# Autodesk Inventor assembly: nano shield
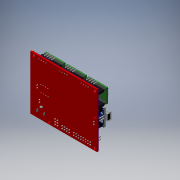
[picture p0: Inventor's stored thumbnail of the model, 180x180]
Saved by Autodesk Inventor 2018 (Build 220112000, 112)
## iProperties
Created: 2018-03-19
Part Number: nano shield
Material: Genérico
Document SubType Name: Assembly
Designer: usuario
Author: usuario
## Documents named in this file (11)
- D:\vape\modelos vape\nano arduino shield cnc\nano shield.iam
- D:\vape\modelos vape\cnc\nano.ipt
- D:\vape\modelos vape\cnc\Headers Machos\Files Inventor\PZ_header_single_1pin.ipt
- D:\vape\modelos vape\cnc\Headers Machos\Files Inventor\PZ_header14pines.ipt
- D:\vape\modelos vape\cnc\Headers Machos\Files Inventor\PZ_header_single_3pines.ipt
- D:\vape\modelos vape\cnc\Headers Machos\Files Inventor\User Library-Header 4 Vertical.ipt
- D:\vape\modelos vape\cnc\arduino-diecimila-t8730\Arduino Diecimila T8730\2.1mm DC Power Socket\2.1mm DC Power Socket.iam
- D:\vape\modelos vape\cnc\arduino-diecimila-t8730\Arduino Diecimila T8730\2.5mm Pitch Miniature Socket - Digital.ipt
- D:\vape\modelos vape\cnc\pololu.ipt
- D:\vape\modelos vape\cnc\SIL_Socket08_.iam
- D:\vape\modelos vape\cnc\arduino-nano-4.snapshot.1\Arduino Nano\Arduino Nano.ipt
## Components (34 placed, 10 different names)
1. nano:1 — Coincidencia:1, Coincidencia:2, Coincidencia:4, Coincidencia:7, Coincidencia:8, Coincidencia:10, Coincidencia:12, Coincidencia:15, Coincidencia:16, Coincidencia:18, Coincidencia:19, Nivelación:7, Coincidencia:20, Coincidencia:21, Coincidencia:25, Coincidencia:26, Coincidencia:27, Coincidencia:28, Coincidencia:29, Coincidencia:30, Coincidencia:31, Coincidencia:32, Coincidencia:33, Coincidencia:37, Coincidencia:39
2. PZ_header_single_1pin:1 — Coincidencia:1, Coincidencia:3, Nivelación:1, Coincidencia:5
3. PZ_header14pines:1 — Coincidencia:2, Coincidencia:3, Nivelación:1, Coincidencia:6, Nivelación:2
4. PZ_header_single_1pin:2 — Coincidencia:4, Coincidencia:5, Coincidencia:6
5. PZ_header_single_1pin:3 — Coincidencia:7, Nivelación:2, Coincidencia:9, Nivelación:3, Coincidencia:14
6. PZ_header_single_1pin:4 — Coincidencia:12, Coincidencia:13, Coincidencia:14
7. PZ_header_single_3pines:1 — Coincidencia:8, Coincidencia:9, Nivelación:3, Coincidencia:11, Nivelación:4, Nivelación:5
8. PZ_header_single_3pines:2 — Coincidencia:10, Coincidencia:11, Nivelación:4, Coincidencia:13
9. PZ_header_single_3pines:3 — Coincidencia:15, Nivelación:5, Nivelación:6, Coincidencia:17
10. PZ_header_single_3pines:4 — Coincidencia:16, Nivelación:6, Coincidencia:17
11. User Library-Header 4 Vertical:1
12. User Library-Header 4 Vertical:2
13. User Library-Header 4 Vertical:3
14. User Library-Header 4 Vertical:4
15. User Library-Header 4 Vertical:5
16. 2.1mm DC Power Socket:1 [sub-assembly] — Coincidencia:18
17. 2.5mm Pitch Miniature Socket - Digital:1 — Coincidencia:19, Nivelación:7, Nivelación:8, Coincidencia:24, Nivelación:14, Nivelación:15
18. 2.5mm Pitch Miniature Socket - Digital:2 — Coincidencia:20, Nivelación:8, Nivelación:9, Coincidencia:23, Nivelación:12, Nivelación:13
19. 2.5mm Pitch Miniature Socket - Digital:3 — Coincidencia:21, Nivelación:9, Coincidencia:22, Nivelación:10, Nivelación:11
20. pololu:1 — Coincidencia:24, Nivelación:14, Nivelación:15, Nivelación:20, Nivelación:21
21. pololu:2 — Coincidencia:23, Nivelación:12, Nivelación:13, Nivelación:18, Nivelación:19
22. pololu:3 — Coincidencia:22, Nivelación:10, Nivelación:11, Nivelación:16, Nivelación:17
23. 2.5mm Pitch Miniature Socket - Digital:4 — Coincidencia:25, Nivelación:16, Nivelación:17
24. 2.5mm Pitch Miniature Socket - Digital:5 — Coincidencia:26, Nivelación:18, Nivelación:19
25. 2.5mm Pitch Miniature Socket - Digital:6 — Coincidencia:27, Nivelación:20, Nivelación:21
26. PZ_header_single_1pin:5 — Coincidencia:31, Coincidencia:34, Nivelación:22
27. PZ_header_single_1pin:6 — Coincidencia:30, Coincidencia:34, Nivelación:22
28. PZ_header_single_1pin:7 — Coincidencia:28, Nivelación:23, Coincidencia:35
29. PZ_header_single_1pin:8 — Coincidencia:29, Nivelación:23, Coincidencia:35
30. PZ_header_single_1pin:9 — Coincidencia:32, Coincidencia:36, Nivelación:24
31. PZ_header_single_1pin:10 — Coincidencia:33, Coincidencia:36, Nivelación:24
32. SIL_Socket08_:1 [sub-assembly] — Coincidencia:37, Coincidencia:38, Nivelación:25, Nivelación:26
33. SIL_Socket08_:2 [sub-assembly] — Coincidencia:39, Nivelación:27, Nivelación:28
34. Arduino Nano:1 — Coincidencia:38, Nivelación:25, Nivelación:26, Nivelación:27, Nivelación:28
## Relationships (67: Mate 39, Flush 28)
- Coincidencia:1 [Mate]: nano:1 ↔ PZ_header_single_1pin:1
- Coincidencia:2 [Mate]: nano:1 ↔ PZ_header14pines:1
- Coincidencia:3 [Mate]: PZ_header_single_1pin:1 ↔ PZ_header14pines:1
- Nivelación:1 [Flush]: PZ_header_single_1pin:1 ↔ PZ_header14pines:1
- Coincidencia:4 [Mate]: nano:1 ↔ PZ_header_single_1pin:2
- Coincidencia:5 [Mate]: PZ_header_single_1pin:1 ↔ PZ_header_single_1pin:2
- Coincidencia:6 [Mate]: PZ_header14pines:1 ↔ PZ_header_single_1pin:2
- Coincidencia:7 [Mate]: nano:1 ↔ PZ_header_single_1pin:3
- Nivelación:2 [Flush]: PZ_header14pines:1 ↔ PZ_header_single_1pin:3
- Coincidencia:8 [Mate]: nano:1 ↔ PZ_header_single_3pines:1
- Coincidencia:9 [Mate]: PZ_header_single_1pin:3 ↔ PZ_header_single_3pines:1
- Nivelación:3 [Flush]: PZ_header_single_1pin:3 ↔ PZ_header_single_3pines:1
- Coincidencia:10 [Mate]: nano:1 ↔ PZ_header_single_3pines:2
- Coincidencia:11 [Mate]: PZ_header_single_3pines:1 ↔ PZ_header_single_3pines:2
- Nivelación:4 [Flush]: PZ_header_single_3pines:1 ↔ PZ_header_single_3pines:2
- Coincidencia:12 [Mate]: nano:1 ↔ PZ_header_single_1pin:4
- Coincidencia:13 [Mate]: PZ_header_single_1pin:4 ↔ PZ_header_single_3pines:2
- Coincidencia:14 [Mate]: PZ_header_single_1pin:3 ↔ PZ_header_single_1pin:4
- Coincidencia:15 [Mate]: nano:1 ↔ PZ_header_single_3pines:3
- Nivelación:5 [Flush]: PZ_header_single_3pines:1 ↔ PZ_header_single_3pines:3
- Coincidencia:16 [Mate]: nano:1 ↔ PZ_header_single_3pines:4
- Nivelación:6 [Flush]: PZ_header_single_3pines:3 ↔ PZ_header_single_3pines:4
- Coincidencia:17 [Mate]: PZ_header_single_3pines:3 ↔ PZ_header_single_3pines:4
- Coincidencia:18 [Mate]: nano:1 ↔ 2.1mm DC Power Socket:1
- Coincidencia:19 [Mate]: nano:1 ↔ 2.5mm Pitch Miniature Socket - Digital:1
- Nivelación:7 [Flush] (2.5 mm): nano:1 ↔ 2.5mm Pitch Miniature Socket - Digital:1
- Coincidencia:20 [Mate]: nano:1 ↔ 2.5mm Pitch Miniature Socket - Digital:2
- Nivelación:8 [Flush]: 2.5mm Pitch Miniature Socket - Digital:1 ↔ 2.5mm Pitch Miniature Socket - Digital:2
- Coincidencia:21 [Mate]: nano:1 ↔ 2.5mm Pitch Miniature Socket - Digital:3
- Nivelación:9 [Flush]: 2.5mm Pitch Miniature Socket - Digital:2 ↔ 2.5mm Pitch Miniature Socket - Digital:3
- Coincidencia:22 [Mate]: 2.5mm Pitch Miniature Socket - Digital:3 ↔ pololu:3
- Nivelación:10 [Flush]: 2.5mm Pitch Miniature Socket - Digital:3 ↔ pololu:3
- Nivelación:11 [Flush]: 2.5mm Pitch Miniature Socket - Digital:3 ↔ pololu:3
- Coincidencia:23 [Mate]: 2.5mm Pitch Miniature Socket - Digital:2 ↔ pololu:2
- Nivelación:12 [Flush]: 2.5mm Pitch Miniature Socket - Digital:2 ↔ pololu:2
- Nivelación:13 [Flush]: 2.5mm Pitch Miniature Socket - Digital:2 ↔ pololu:2
- Coincidencia:24 [Mate]: 2.5mm Pitch Miniature Socket - Digital:1 ↔ pololu:1
- Nivelación:14 [Flush]: 2.5mm Pitch Miniature Socket - Digital:1 ↔ pololu:1
- Nivelación:15 [Flush]: 2.5mm Pitch Miniature Socket - Digital:1 ↔ pololu:1
- Coincidencia:25 [Mate]: nano:1 ↔ 2.5mm Pitch Miniature Socket - Digital:4
- Nivelación:16 [Flush]: pololu:3 ↔ 2.5mm Pitch Miniature Socket - Digital:4
- Nivelación:17 [Flush]: pololu:3 ↔ 2.5mm Pitch Miniature Socket - Digital:4
- Coincidencia:26 [Mate]: nano:1 ↔ 2.5mm Pitch Miniature Socket - Digital:5
- Nivelación:18 [Flush]: pololu:2 ↔ 2.5mm Pitch Miniature Socket - Digital:5
- Nivelación:19 [Flush]: pololu:2 ↔ 2.5mm Pitch Miniature Socket - Digital:5
- Coincidencia:27 [Mate]: nano:1 ↔ 2.5mm Pitch Miniature Socket - Digital:6
- Nivelación:20 [Flush]: pololu:1 ↔ 2.5mm Pitch Miniature Socket - Digital:6
- Nivelación:21 [Flush]: pololu:1 ↔ 2.5mm Pitch Miniature Socket - Digital:6
- Coincidencia:28 [Mate]: nano:1 ↔ PZ_header_single_1pin:7
- Coincidencia:29 [Mate]: nano:1 ↔ PZ_header_single_1pin:8
- Coincidencia:30 [Mate]: nano:1 ↔ PZ_header_single_1pin:6
- Coincidencia:31 [Mate]: nano:1 ↔ PZ_header_single_1pin:5
- Coincidencia:32 [Mate]: nano:1 ↔ PZ_header_single_1pin:9
- Coincidencia:33 [Mate]: nano:1 ↔ PZ_header_single_1pin:10
- Coincidencia:34 [Mate]: PZ_header_single_1pin:5 ↔ PZ_header_single_1pin:6
- Nivelación:22 [Flush]: PZ_header_single_1pin:5 ↔ PZ_header_single_1pin:6
- Nivelación:23 [Flush]: PZ_header_single_1pin:7 ↔ PZ_header_single_1pin:8
- Coincidencia:35 [Mate]: PZ_header_single_1pin:7 ↔ PZ_header_single_1pin:8
- Coincidencia:36 [Mate]: PZ_header_single_1pin:9 ↔ PZ_header_single_1pin:10
- Nivelación:24 [Flush]: PZ_header_single_1pin:9 ↔ PZ_header_single_1pin:10
- Coincidencia:37 [Mate]: nano:1 ↔ SIL_Socket08_:1
- Coincidencia:38 [Mate]: SIL_Socket08_:1 ↔ Arduino Nano:1
- Nivelación:25 [Flush]: SIL_Socket08_:1 ↔ Arduino Nano:1
- Nivelación:26 [Flush]: SIL_Socket08_:1 ↔ Arduino Nano:1
- Coincidencia:39 [Mate]: nano:1 ↔ SIL_Socket08_:2
- Nivelación:27 [Flush]: SIL_Socket08_:2 ↔ Arduino Nano:1
- Nivelación:28 [Flush]: SIL_Socket08_:2 ↔ Arduino Nano:1
